# Autodesk Inventor assembly: Speaker_Box
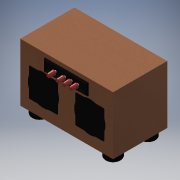
[picture p0: Inventor's stored thumbnail of the model, 180x180]
Saved by Autodesk Inventor 2017 (Build 210142000, 142)
## iProperties
Created: 2019-01-31
Part Number: Speaker_Box
Document SubType Name: Assembly
Designer: Mitch
Author: Mitch
## Documents named in this file (12)
- E:\Youtube Channel\Pojects\Bluetooth Speaker\MECH\Speaker_Box.iam
- E:\Youtube Channel\Pojects\Bluetooth Speaker\MECH\Bottom.ipt
- E:\Youtube Channel\Pojects\Bluetooth Speaker\MECH\Front.ipt
- E:\Youtube Channel\Pojects\Bluetooth Speaker\MECH\Right Side.ipt
- E:\Youtube Channel\Pojects\Bluetooth Speaker\MECH\Left Side.ipt
- E:\Youtube Channel\Pojects\Bluetooth Speaker\MECH\Back.ipt
- E:\Youtube Channel\Pojects\Bluetooth Speaker\MECH\Top.ipt
- E:\Youtube Channel\Pojects\Bluetooth Speaker\MECH\4in_speaker.ipt
- E:\Youtube Channel\Pojects\Bluetooth Speaker\MECH\sub.ipt
- E:\Youtube Channel\Pojects\Bluetooth Speaker\MECH\foot.ipt
- E:\Youtube Channel\Pojects\Bluetooth Speaker\MECH\Amplifier Assembly.iam
- E:\Youtube Channel\Pojects\Bluetooth Speaker\MECH\chroma cap.ipt
## Components (18 placed, 11 different names)
1. Bottom:1 — Mate:1, Flush:1, Flush:2, Flush:3, Mate:2, Flush:4, Mate:5, Mate:6, Flush:6, Mate:19, Mate:20, Mate:21, Mate:22, Mate:23, Mate:24, Tangent:1, Tangent:2, Tangent:3, Tangent:4, Tangent:5, Tangent:6, Tangent:7, Tangent:8
2. Front:1 — Mate:1, Flush:1, Flush:2, Mate:3, Mate:4, Flush:8, Mate:15, Mate:16, Mate:17, Mate:18, Mate:27
3. Right Side:1 — Flush:4, Mate:4, Mate:5, Flush:5, Mate:7, Flush:7
4. Left Side:1 — Flush:3, Mate:2, Mate:3, Mate:26
5. Back:1 — Mate:6, Flush:5, Flush:6
6. Top:1 — Mate:7, Flush:7, Flush:8, Mate:25
7. 4in_speaker:1 — Mate:15, Mate:17
8. 4in_speaker:2 — Mate:16, Mate:18
9. sub:1 — Mate:19, Mate:20
10. foot:1 — Mate:21, Tangent:5, Tangent:6
11. foot:2 — Mate:23, Tangent:3, Tangent:4
12. foot:3 — Mate:22, Tangent:7, Tangent:8
13. foot:4 — Mate:24, Tangent:1, Tangent:2
14. Amplifier Assembly:1 [sub-assembly] — Mate:25, Mate:26, Mate:27, Mate:28, Mate:29, Mate:30, Mate:31, Mate:32, Mate:33, Mate:34, Mate:35
15. chroma cap:1 — Mate:28, Mate:32
16. chroma cap:2 — Mate:29, Mate:33
17. chroma cap:3 — Mate:30, Mate:34
18. chroma cap:4 — Mate:31, Mate:35
## Relationships (44: Mate 28, Flush 8, Tangent 8)
- Mate:1: Bottom:1 ↔ Front:1
- Flush:1: Bottom:1 ↔ Front:1
- Flush:2: Bottom:1 ↔ Front:1
- Flush:3: Bottom:1 ↔ Left Side:1
- Mate:2: Bottom:1 ↔ Left Side:1
- Mate:3: Front:1 ↔ Left Side:1
- Flush:4: Bottom:1 ↔ Right Side:1
- Mate:4: Front:1 ↔ Right Side:1
- Mate:5: Bottom:1 ↔ Right Side:1
- Mate:6: Bottom:1 ↔ Back:1
- Flush:5: Right Side:1 ↔ Back:1
- Flush:6: Bottom:1 ↔ Back:1
- Mate:7: Right Side:1 ↔ Top:1
- Flush:7: Right Side:1 ↔ Top:1
- Flush:8: Front:1 ↔ Top:1
- Mate:15: Front:1 ↔ 4in_speaker:1
- Mate:16: Front:1 ↔ 4in_speaker:2
- Mate:17: Front:1 ↔ 4in_speaker:1
- Mate:18: Front:1 ↔ 4in_speaker:2
- Mate:19: Bottom:1 ↔ sub:1
- Mate:20: Bottom:1 ↔ sub:1
- Mate:21: Bottom:1 ↔ foot:1
- Mate:22: Bottom:1 ↔ foot:3
- Mate:23: Bottom:1 ↔ foot:2
- Mate:24: Bottom:1 ↔ foot:4
- Tangent:1 (-57.15 mm): Bottom:1 ↔ foot:4
- Tangent:2 (-57.15 mm): Bottom:1 ↔ foot:4
- Tangent:3 (-57.15 mm): Bottom:1 ↔ foot:2
- Tangent:4 (-57.15 mm): Bottom:1 ↔ foot:2
- Tangent:5 (-57.15 mm): Bottom:1 ↔ foot:1
- Tangent:6 (-57.15 mm): Bottom:1 ↔ foot:1
- Tangent:7 (-57.15 mm): Bottom:1 ↔ foot:3
- Tangent:8 (-57.15 mm): Bottom:1 ↔ foot:3
- Mate:25: Top:1 ↔ Amplifier Assembly:1
- Mate:26 (67.945 mm): Left Side:1 ↔ Amplifier Assembly:1
- Mate:27: Front:1 ↔ Amplifier Assembly:1
- Mate:28: Amplifier Assembly:1 ↔ chroma cap:1
- Mate:29: Amplifier Assembly:1 ↔ chroma cap:2
- Mate:30: Amplifier Assembly:1 ↔ chroma cap:3
- Mate:31: Amplifier Assembly:1 ↔ chroma cap:4
- Mate:32 (5.08 mm): Amplifier Assembly:1 ↔ chroma cap:1
- Mate:33 (5.08 mm): Amplifier Assembly:1 ↔ chroma cap:2
- Mate:34 (5.08 mm): Amplifier Assembly:1 ↔ chroma cap:3
- Mate:35 (5.08 mm): Amplifier Assembly:1 ↔ chroma cap:4
